# Autodesk Inventor assembly: Bumper Attachment 2
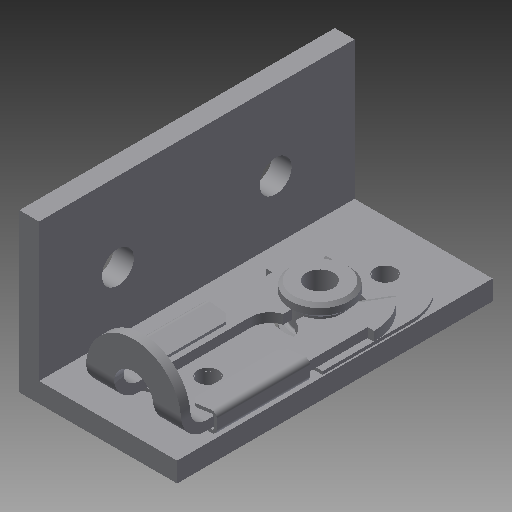
[picture p0: Inventor's stored thumbnail of the model, 512x512]
Saved by Autodesk Inventor 2018 (Build 220112000, 112)
## iProperties
Created: 2020-01-24
Part Number: Bumper Attachment 2
Document SubType Name: Assembly
Designer: S-2512711
Author: S-2512711
## Documents named in this file (3)
- C:\Users\maste\OneDrive\Documents\GitHub\2020CAD\Bumpers\Part Files\Bumper Attachment 2.iam
- C:\Users\maste\OneDrive\Documents\GitHub\2020CAD\Bumpers\Part Files\2in L-Bracket 2.ipt
- C:\Users\maste\OneDrive\Documents\GitHub\2020CAD\Bumpers\Part Files\1872A720_SLIDE-SNAP DRAW LATCH.ipt
## Components (2 placed, 2 different names)
1. 2in L-Bracket 2:1 — Mate:1, Mate:2, Rotation:1
2. 1872A720_SLIDE-SNAP DRAW LATCH:1 — Mate:1, Mate:2, Rotation:1
## Relationships (3: Mate 2, RelateRotation 1)
- Mate:1: 2in L-Bracket 2:1 ↔ 1872A720_SLIDE-SNAP DRAW LATCH:1
- Mate:2: 2in L-Bracket 2:1 ↔ 1872A720_SLIDE-SNAP DRAW LATCH:1
- Rotation:1 [RelateRotation] (1 ul): 2in L-Bracket 2:1 ↔ 1872A720_SLIDE-SNAP DRAW LATCH:1
